# Autodesk Inventor assembly: Polycarb main conv
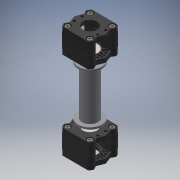
[picture p0: Inventor's stored thumbnail of the model, 180x180]
Saved by Autodesk Inventor 2018 (Build 220112000, 112)
## iProperties
Created: 2020-01-27
Part Number: Polycarb main conv
Document SubType Name: Assembly
Designer: Burni
Author: Burni
## Documents named in this file (5)
- \\studenthome\students\S-4008082\GitHub\2020CAD\Tyler's Ball Storage\Polycarb half main conv.iam
- \\studenthome\students\S-4008082\GitHub\2020CAD\Tyler's Ball Storage\Hex shaft\Shooter hex shaft.ipt
- \\studenthome\students\S-4008082\GitHub\2020CAD\Tyler's Ball Storage\Other parts\Polycord conveyor.ipt
- \\studenthome\students\S-4008082\GitHub\2020CAD\Tyler's Ball Storage\Other parts\VersaBlock_Mini_Kit_217-5852.iam
- \\studenthome\students\S-4008082\GitHub\2020CAD\Tyler's Ball Storage\Other parts\am-0028 00.375'' id Flanged, Shielded Ball Bearing (FR6ZZ).ipt
## Components (6 placed, 4 different names)
1. Shooter hex shaft:1 — Mate:33, Mate:34, Flush:1, Flush:2
2. Polycord conveyor:1 — Mate:33, Mate:34, Flush:1, Mate:43
3. VersaBlock_Mini_Kit_217-5852:1 [sub-assembly] — Mate:38, Mate:39, Mate:40, Mate:42
4. VersaBlock_Mini_Kit_217-5852:2 [sub-assembly] — Mate:36, Mate:37, Mate:40, Mate:42
5. am-0028 00.375'' id Flanged, Shielded Ball Bearing (FR6ZZ):3 — Mate:36, Mate:37, Mate:41
6. am-0028 00.375'' id Flanged, Shielded Ball Bearing (FR6ZZ):4 — Mate:38, Mate:39, Mate:41, Mate:43, Flush:2
## Relationships (12: Mate 10, Flush 2)
- Mate:33: Shooter hex shaft:1 ↔ Polycord conveyor:1
- Mate:34: Shooter hex shaft:1 ↔ Polycord conveyor:1
- Flush:1 (16.0655 mm): Shooter hex shaft:1 ↔ Polycord conveyor:1
- Mate:36: VersaBlock_Mini_Kit_217-5852:2 ↔ am-0028 00.375'' id Flanged, Shielded Ball Bearing (FR6ZZ):3
- Mate:37: VersaBlock_Mini_Kit_217-5852:2 ↔ am-0028 00.375'' id Flanged, Shielded Ball Bearing (FR6ZZ):3
- Mate:38: VersaBlock_Mini_Kit_217-5852:1 ↔ am-0028 00.375'' id Flanged, Shielded Ball Bearing (FR6ZZ):4
- Mate:39: VersaBlock_Mini_Kit_217-5852:1 ↔ am-0028 00.375'' id Flanged, Shielded Ball Bearing (FR6ZZ):4
- Mate:40 (101.6 mm): VersaBlock_Mini_Kit_217-5852:1 ↔ VersaBlock_Mini_Kit_217-5852:2
- Mate:41: am-0028 00.375'' id Flanged, Shielded Ball Bearing (FR6ZZ):3 ↔ am-0028 00.375'' id Flanged, Shielded Ball Bearing (FR6ZZ):4
- Mate:42: VersaBlock_Mini_Kit_217-5852:1 ↔ VersaBlock_Mini_Kit_217-5852:2
- Mate:43: Polycord conveyor:1 ↔ am-0028 00.375'' id Flanged, Shielded Ball Bearing (FR6ZZ):4
- Flush:2: Shooter hex shaft:1 ↔ am-0028 00.375'' id Flanged, Shielded Ball Bearing (FR6ZZ):4
